# Autodesk Inventor assembly: conjunto engranajes dimer, hombro y codo
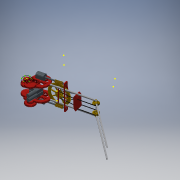
[picture p0: Inventor's stored thumbnail of the model, 180x180]
Saved by Autodesk Inventor 2016 (Build 200138000, 138)
## iProperties
Created: 2016-06-23
Part Number: conjunto engranajes dimer, hombro y codo
Document SubType Name: Assembly
Designer: Admin
Author: Admin
## Documents named in this file (15)
- C:\Users\Admin\Dropbox\diseños autodesk dimer\conjunto engranajes dimer, hombro y codo.iam
- C:\Users\Admin\Dropbox\diseños autodesk dimer\engranajes dimer hombro muelles\engranaje gusano.ipt
- C:\Users\Admin\Dropbox\diseños autodesk dimer\engranajes dimer hombro muelles\engranajes motor hombro dimer 3.1.iam
- C:\Users\Admin\Dropbox\diseños autodesk dimer\engranajes dimer hombro muelles\engranajes motor hombro dimer 3.1_MIR2.iam
- C:\Users\Admin\Dropbox\diseños autodesk dimer\ENGRANAJES GUSANO BRAZO COPIA SEGURIDAD 30.7.iam
- C:\Users\Admin\Dropbox\diseños autodesk dimer\engrane gusano horizonatal taladro.iam
- C:\Users\Admin\Dropbox\diseños autodesk dimer\taladro.ipt
- C:\Users\Admin\Dropbox\diseños autodesk dimer\eje codo.ipt
- C:\Users\Admin\Dropbox\diseños autodesk dimer\engranajes dimer hombro muelles\perfil aluminio.ipt
- C:\Users\Admin\Dropbox\diseños autodesk dimer\enganche correa codo.iam
- C:\Users\Admin\Dropbox\diseños autodesk dimer\motor hombro.ipt
- C:\Users\Admin\Dropbox\diseños autodesk dimer\estructura union gusano.ipt
- C:\Users\Admin\Dropbox\diseños autodesk dimer\enganche vertical rueda gusano.ipt
- C:\Users\Admin\Documents\piezas 3d dimer\engranajes motor hombro dimer 3.1\correa codo.ipt
- C:\Users\Admin\Documents\piezas 3d dimer\engranajes motor hombro dimer 3.1\giro 90º correa.ipt
## Components (22 placed, 14 different names)
1. engranaje gusano:1
2. engranajes motor hombro dimer 3.1:1 [sub-assembly] — Mate:1, Flush:1, Mate:2, Mate:4, Mate:8, Flush:8, Mate:14
3. engranajes motor hombro dimer 3.1_MIR2:1 [sub-assembly] — Mate:1, Flush:1, Mate:2, Flush:7, Flush:9, Mate:11, Mate:15, Flush:16, Mate:23, Flush:23
4. ENGRANAJES GUSANO BRAZO COPIA SEGURIDAD 30.7:1 [sub-assembly] — Mate:4, Mate:27, Mate:28, Mate:30, Mate:32, Flush:22
5. engrane gusano horizonatal taladro:1 [sub-assembly] — Flush:3
6. engrane gusano horizonatal taladro:2 [sub-assembly] — Flush:3
7. taladro:1 — Flush:6, Mate:24, Mate:25
8. taladro:2 — Mate:8, Flush:6, Mate:31
9. eje codo:1 — Flush:7, Flush:8, Flush:9, Mate:15, Mate:16
10. perfil aluminio:1 — Mate:11, Flush:10, Flush:11, Mate:20, Mate:21
11. perfil aluminio:2 — Flush:10, Mate:14, Mate:16, Flush:11, Mate:19, Flush:12
12. Spur Gears:1 [sub-assembly] — Mate:19, Flush:12, Flush:13, Flush:17, Flush:19, Flush:21
13. Spur Gears:2 [sub-assembly] — Flush:13, Mate:20, Mate:21, Mate:29
14. motor hombro:1 — Mate:22, Flush:14, Flush:15, Flush:16, Mate:23
15. motor hombro:2 — Mate:22, Flush:14, Flush:15
16. estructura union gusano:1 — Mate:24, Mate:25, Flush:18, Flush:20, Mate:31
17. enganche vertical rueda gusano:1 — Mate:27, Mate:28
18. correa codo:1 — Flush:17, Flush:18, Flush:19, Flush:20, Flush:21
19. correa codo:2 — Mate:29
20. correa codo:3 — Mate:30
21. correa codo:4 — Mate:32
22. giro 90º correa:1 — Flush:22, Flush:23
## Relationships (41: Mate 21, Flush 20)
- Mate:1: engranajes motor hombro dimer 3.1:1 ↔ engranajes motor hombro dimer 3.1_MIR2:1
- Flush:1: engranajes motor hombro dimer 3.1:1 ↔ engranajes motor hombro dimer 3.1_MIR2:1
- Mate:2 (132 mm): engranajes motor hombro dimer 3.1:1 ↔ engranajes motor hombro dimer 3.1_MIR2:1
- Mate:4 (1 mm): engranajes motor hombro dimer 3.1:1 ↔ ENGRANAJES GUSANO BRAZO COPIA SEGURIDAD 30.7:1
- Flush:3: engrane gusano horizonatal taladro:1 ↔ engrane gusano horizonatal taladro:2
- Mate:8: engranajes motor hombro dimer 3.1:1 ↔ taladro:2
- Flush:6: taladro:1 ↔ taladro:2
- Flush:7: engranajes motor hombro dimer 3.1_MIR2:1 ↔ eje codo:1
- Flush:8: engranajes motor hombro dimer 3.1:1 ↔ eje codo:1
- Flush:9: engranajes motor hombro dimer 3.1_MIR2:1 ↔ eje codo:1
- Mate:11 (4 mm): engranajes motor hombro dimer 3.1_MIR2:1 ↔ perfil aluminio:1
- Flush:10: perfil aluminio:1 ↔ perfil aluminio:2
- Mate:14 (4 mm): engranajes motor hombro dimer 3.1:1 ↔ perfil aluminio:2
- Mate:15: engranajes motor hombro dimer 3.1_MIR2:1 ↔ eje codo:1
- Mate:16: eje codo:1 ↔ perfil aluminio:2
- Flush:11: perfil aluminio:1 ↔ perfil aluminio:2
- Mate:19 (0.5 mm): perfil aluminio:2 ↔ Spur Gears:1
- Flush:12 (-19 mm): perfil aluminio:2 ↔ Spur Gears:1
- Flush:13: Spur Gears:1 ↔ Spur Gears:2
- Mate:20 (0.5 mm): perfil aluminio:1 ↔ Spur Gears:2
- Mate:21 (0.5 mm): perfil aluminio:1 ↔ Spur Gears:2
- Mate:22 (7 mm): motor hombro:1 ↔ motor hombro:2
- Flush:14: motor hombro:1 ↔ motor hombro:2
- Flush:15: motor hombro:1 ↔ motor hombro:2
- Flush:16 (-13 mm): engranajes motor hombro dimer 3.1_MIR2:1 ↔ motor hombro:1
- Mate:23: engranajes motor hombro dimer 3.1_MIR2:1 ↔ motor hombro:1
- Mate:24: taladro:1 ↔ estructura union gusano:1
- Mate:25: taladro:1 ↔ estructura union gusano:1
- Mate:27: ENGRANAJES GUSANO BRAZO COPIA SEGURIDAD 30.7:1 ↔ enganche vertical rueda gusano:1
- Mate:28: ENGRANAJES GUSANO BRAZO COPIA SEGURIDAD 30.7:1 ↔ enganche vertical rueda gusano:1
- Flush:17: Spur Gears:1 ↔ correa codo:1
- Flush:18: estructura union gusano:1 ↔ correa codo:1
- Flush:19: Spur Gears:1 ↔ correa codo:1
- Flush:20: estructura union gusano:1 ↔ correa codo:1
- Flush:21: Spur Gears:1 ↔ correa codo:1
- Mate:29: Spur Gears:2 ↔ correa codo:2
- Mate:30: ENGRANAJES GUSANO BRAZO COPIA SEGURIDAD 30.7:1 ↔ correa codo:3
- Mate:31: taladro:2 ↔ estructura union gusano:1
- Mate:32: ENGRANAJES GUSANO BRAZO COPIA SEGURIDAD 30.7:1 ↔ correa codo:4
- Flush:22: ENGRANAJES GUSANO BRAZO COPIA SEGURIDAD 30.7:1 ↔ giro 90º correa:1
- Flush:23: engranajes motor hombro dimer 3.1_MIR2:1 ↔ giro 90º correa:1
